# Autodesk Inventor assembly: Calosc
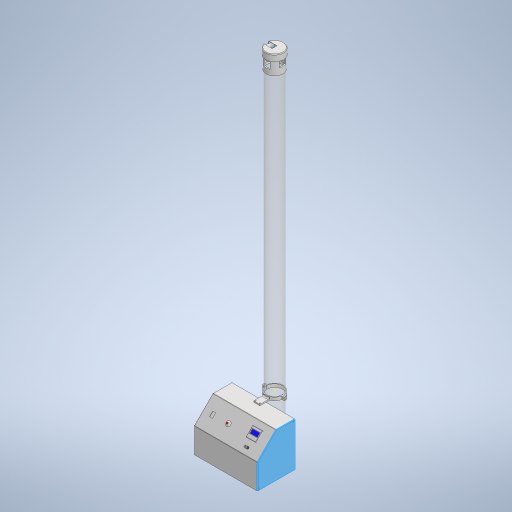
[picture p0: Inventor's stored thumbnail of the model, 512x512]
Saved by Autodesk Inventor 2024.3 (Build 283343000, 343)
## iProperties
Created: 2024-12-26
Part Number: Calosc
Document SubType Name: Assembly
Designer: adamn
Author: adamn
## Documents named in this file (15)
- C:\Users\adamn\Desktop\ProjektSTM\Calosc.iam
- C:\Users\adamn\Desktop\ProjektSTM\PanelGlowny.ipt
- C:\Users\adamn\Desktop\ProjektSTM\PodstawaRury.ipt
- C:\Users\adamn\Desktop\ProjektSTM\Rura.ipt
- C:\Users\adamn\Desktop\ProjektSTM\led-red-5mm-2.snapshot.1\BTG_901_BT_001_LED_5mm_Rot\LED_5mm_Rot.ipt
- C:\Users\adamn\Desktop\ProjektSTM\enkoder.ipt
- C:\Users\adamn\Desktop\ProjektSTM\oled_096_gm009605.ipt
- C:\Users\adamn\Desktop\ProjektSTM\50-mm-dc-fan-1.snapshot.2\JAMICO FAN 50X50X10.ipt
- C:\Users\adamn\Desktop\ProjektSTM\MocowanieBoku.ipt
- C:\Users\adamn\Desktop\ProjektSTM\PanelBoczny.ipt
- C:\Users\adamn\Desktop\ProjektSTM\UchwytRuryGlowny.ipt
- C:\Users\adamn\Desktop\ProjektSTM\OpaskaRury.ipt
- C:\Users\adamn\Desktop\ProjektSTM\CzujnikUltraDziekowy.iam
- C:\Users\adamn\Desktop\ProjektSTM\OslonaLED.ipt
- C:\Users\adamn\Desktop\ProjektSTM\OslonaWyswietlacza.ipt
## Components (15 placed, 14 different names)
1. PanelGlowny:1 — Zestawiające:1, Wstawiające:1, Wstawiające:2, Zestawiające:3, Zestawiające:4, Zestawiające:5, Zestawiające:6, Zestawiające:7, Zestawiające:8, Zestawiające:9, Zestawiające:10, Zestawiające:13, Zestawiające:14, Zestawiające:15, Zestawiające:16, Zestawiające:17, Zestawiające:18, Wstawiające:6, Wstawiające:7
2. PodstawaRury:1 — Zestawiające:1, Wstawiające:1, Wstawiające:2, Zestawiające:2, Zestawiające:11, Zestawiające:12, Wstawiające:3
3. Rura:1 — Zestawiające:2, Wstawiające:10
4. LED_5mm_Rot:1 — Zestawiające:3, Zestawiające:4, Zestawiające:5, Wstawiające:11
5. enkoder:1 — Zestawiające:6, Zestawiające:7
6. oled_096_gm009605:1 — Zestawiające:8, Zestawiające:9, Zestawiające:10, Zestawiające:19, Zestawiające:20
7. JAMICO FAN 50X50X10:1 — Zestawiające:11, Zestawiające:12, Wstawiające:3
8. MocowanieBoku:1 — Zestawiające:13, Zestawiające:14, Zestawiające:15, Wstawiające:4
9. MocowanieBoku:2 — Zestawiające:16, Zestawiające:17, Zestawiające:18, Wstawiające:5
10. PanelBoczny:1 — Wstawiające:4, Wstawiające:5
11. UchwytRuryGlowny:1 — Wstawiające:6, Wstawiające:7, Wstawiające:8, Wstawiające:9
12. OpaskaRury:1 — Wstawiające:8, Wstawiające:9
13. CzujnikUltraDziekowy:1 [sub-assembly] — Wstawiające:10
14. OslonaLED:1 — Wstawiające:11
15. OslonaWyswietlacza:1 — Zestawiające:19, Zestawiające:20
## Relationships (31: Mate 20, Insert 11)
- Zestawiające:1 [Mate]: PanelGlowny:1 ↔ PodstawaRury:1
- Wstawiające:1 [Insert]: PanelGlowny:1 ↔ PodstawaRury:1
- Wstawiające:2 [Insert]: PanelGlowny:1 ↔ PodstawaRury:1
- Zestawiające:2 [Mate]: PodstawaRury:1 ↔ Rura:1
- Zestawiające:3 [Mate]: PanelGlowny:1 ↔ LED_5mm_Rot:1
- Zestawiające:4 [Mate] (1 mm): PanelGlowny:1 ↔ LED_5mm_Rot:1
- Zestawiające:5 [Mate] (1 mm): PanelGlowny:1 ↔ LED_5mm_Rot:1
- Zestawiające:6 [Mate]: PanelGlowny:1 ↔ enkoder:1
- Zestawiające:7 [Mate]: PanelGlowny:1 ↔ enkoder:1
- Zestawiające:8 [Mate]: PanelGlowny:1 ↔ oled_096_gm009605:1
- Zestawiające:9 [Mate]: PanelGlowny:1 ↔ oled_096_gm009605:1
- Zestawiające:10 [Mate]: PanelGlowny:1 ↔ oled_096_gm009605:1
- Zestawiające:11 [Mate]: PodstawaRury:1 ↔ JAMICO FAN 50X50X10:1
- Zestawiające:12 [Mate]: PodstawaRury:1 ↔ JAMICO FAN 50X50X10:1
- Wstawiające:3 [Insert]: PodstawaRury:1 ↔ JAMICO FAN 50X50X10:1
- Zestawiające:13 [Mate]: PanelGlowny:1 ↔ MocowanieBoku:1
- Zestawiające:14 [Mate]: PanelGlowny:1 ↔ MocowanieBoku:1
- Zestawiające:15 [Mate]: PanelGlowny:1 ↔ MocowanieBoku:1
- Zestawiające:16 [Mate]: PanelGlowny:1 ↔ MocowanieBoku:2
- Zestawiające:17 [Mate]: PanelGlowny:1 ↔ MocowanieBoku:2
- Zestawiające:18 [Mate]: PanelGlowny:1 ↔ MocowanieBoku:2
- Wstawiające:4 [Insert]: MocowanieBoku:1 ↔ PanelBoczny:1
- Wstawiające:5 [Insert]: MocowanieBoku:2 ↔ PanelBoczny:1
- Wstawiające:6 [Insert]: PanelGlowny:1 ↔ UchwytRuryGlowny:1
- Wstawiające:7 [Insert]: PanelGlowny:1 ↔ UchwytRuryGlowny:1
- Wstawiające:8 [Insert]: UchwytRuryGlowny:1 ↔ OpaskaRury:1
- Wstawiające:9 [Insert]: UchwytRuryGlowny:1 ↔ OpaskaRury:1
- Wstawiające:10 [Insert]: Rura:1 ↔ CzujnikUltraDziekowy:1
- Wstawiające:11 [Insert]: LED_5mm_Rot:1 ↔ OslonaLED:1
- Zestawiające:19 [Mate]: oled_096_gm009605:1 ↔ OslonaWyswietlacza:1
- Zestawiające:20 [Mate]: oled_096_gm009605:1 ↔ OslonaWyswietlacza:1
